# Autodesk Inventor assembly: Prototype-Chassis-1
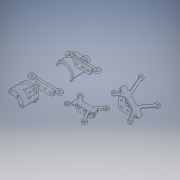
[picture p0: Inventor's stored thumbnail of the model, 180x180]
Saved by Autodesk Inventor 2017 (Build 210142000, 142)
## iProperties
Created: 2018-04-11
Part Number: Prototype-Chassis-1
Document SubType Name: Assembly
Designer: MtgSaber
Author: MtgSaber
## Documents named in this file (12)
- D:\Programming\Projects\Pirover\autodesk\Prototype-Chassis-1.iam
- D:\Programming\Projects\Pirover\autodesk\2.5in-wheel\2.5in-Wheel-2.ipt
- D:\Programming\Projects\Pirover\autodesk\Nextrox-Mini-12VDC-60rpmGearbox-Motor\Nextrox-Mini-12VDC-60rpmGearbox-Motor.ipt
- D:\Programming\Projects\Pirover\autodesk\Keystone-26650-Dual-Battery-Holder\Keystone-26650-Dual-Battery-Holder[DWG-1109].ipt
- D:\Programming\Projects\Pirover\autodesk\Drok-DC-9v+-to-5v-Converter\Drok-DC-9v+-to-5v-Converter.ipt
- D:\Programming\Projects\Pirover\autodesk\Raspberry-Pi-3BPlus[with_Screen]\Raspberry-Pi-3B[with_Screen].ipt
- D:\Programming\Projects\Pirover\autodesk\Arduino-Uno-r3\Arduino-Uno-r3.ipt
- D:\Programming\Projects\Pirover\autodesk\ChasssiPrototypeA2.ipt
- D:\Programming\Projects\Pirover\autodesk\ChasssiPrototypeA2_MIR.ipt
- D:\Programming\Projects\Pirover\autodesk\ChassisPrototypeA3.ipt
- D:\Programming\Projects\Pirover\autodesk\ChassisPrototypeA4.ipt
- D:\Programming\Projects\Pirover\autodesk\ChassisPrototypeA5.ipt
## Components (15 placed, 11 different names)
1. Nextrox-Mini-12VDC-60rpmGearbox-Motor:1 — Mate:2, Mate:3, Mate:9, Flush:11, Flush:15, Mate:17, Mate:18, Mate:20, Mate:21, Mate:22
2. Nextrox-Mini-12VDC-60rpmGearbox-Motor:2 — Mate:2, Mate:3, Flush:10, Flush:14, Mate:15, Mate:16, Mate:19, Flush:16
3. Keystone-26650-Dual-Battery-Holder[DWG-1109]:1 — Mate:5, Flush:2, Flush:3, Mate:6, Flush:7, Flush:8, Mate:7, Flush:11, Flush:12, Mate:23, Mate:24
4. Keystone-26650-Dual-Battery-Holder[DWG-1109]:2 — Mate:5, Flush:2, Flush:3, Flush:6, Flush:10, Mate:19, Flush:17, Flush:18
5. Drok-DC-9v+-to-5v-Converter:1 — Flush:1, Flush:5, Mate:6, Flush:7, Mate:12
6. Raspberry-Pi-3B[with_Screen]:1 — Flush:13, Mate:11, Angle:1, Mate:13, Angle:2, Flush:26, Flush:27
7. Arduino-Uno-r3:1 — Flush:1, Flush:5, Flush:6, Mate:8, Flush:21, Flush:22, Flush:23, Flush:24, Flush:25
8. 2.5in-Wheel-2:1 — Flush:15, Mate:17, Mate:18
9. 2.5in-Wheel-2:2 — Flush:14, Mate:15, Mate:16
10. ChasssiPrototypeA2:1 — Flush:16
11. ChasssiPrototypeA2_MIR:1 — Mate:20, Mate:21, Mate:22
12. ChassisPrototypeA3:1 — Flush:17, Flush:19, Flush:20
13. ChassisPrototypeA3:2 — Mate:23, Flush:20, Mate:24
14. ChassisPrototypeA4:1 — Flush:21, Flush:23, Flush:24, Flush:25
15. ChassisPrototypeA5:1 — Flush:26, Flush:28
## Relationships (49: Flush 26, Mate 21, Angle 2)
- Mate:2: Nextrox-Mini-12VDC-60rpmGearbox-Motor:1 ↔ Nextrox-Mini-12VDC-60rpmGearbox-Motor:2
- Mate:3: Nextrox-Mini-12VDC-60rpmGearbox-Motor:1 ↔ Nextrox-Mini-12VDC-60rpmGearbox-Motor:2
- Flush:1: Drok-DC-9v+-to-5v-Converter:1 ↔ Arduino-Uno-r3:1
- Mate:5 (25.4 mm): Keystone-26650-Dual-Battery-Holder[DWG-1109]:1 ↔ Keystone-26650-Dual-Battery-Holder[DWG-1109]:2
- Flush:2: Keystone-26650-Dual-Battery-Holder[DWG-1109]:1 ↔ Keystone-26650-Dual-Battery-Holder[DWG-1109]:2
- Flush:3: Keystone-26650-Dual-Battery-Holder[DWG-1109]:1 ↔ Keystone-26650-Dual-Battery-Holder[DWG-1109]:2
- Flush:5: Drok-DC-9v+-to-5v-Converter:1 ↔ Arduino-Uno-r3:1
- Mate:6 (25.4 mm): Keystone-26650-Dual-Battery-Holder[DWG-1109]:1 ↔ Drok-DC-9v+-to-5v-Converter:1
- Flush:6: Keystone-26650-Dual-Battery-Holder[DWG-1109]:2 ↔ Arduino-Uno-r3:1
- Flush:7: Keystone-26650-Dual-Battery-Holder[DWG-1109]:1 ↔ Drok-DC-9v+-to-5v-Converter:1
- Flush:8: Keystone-26650-Dual-Battery-Holder[DWG-1109]:1
- Mate:7: Keystone-26650-Dual-Battery-Holder[DWG-1109]:1
- Mate:8: Arduino-Uno-r3:1
- Mate:9 (-38.1 mm): Nextrox-Mini-12VDC-60rpmGearbox-Motor:1
- Flush:10: Nextrox-Mini-12VDC-60rpmGearbox-Motor:2 ↔ Keystone-26650-Dual-Battery-Holder[DWG-1109]:2
- Flush:11: Nextrox-Mini-12VDC-60rpmGearbox-Motor:1 ↔ Keystone-26650-Dual-Battery-Holder[DWG-1109]:1
- Flush:12 (12.7 mm): Keystone-26650-Dual-Battery-Holder[DWG-1109]:1
- Flush:13: Raspberry-Pi-3B[with_Screen]:1
- Mate:11: Raspberry-Pi-3B[with_Screen]:1
- Angle:1 (-45 deg): Raspberry-Pi-3B[with_Screen]:1
- Mate:12 (25.4 mm): Drok-DC-9v+-to-5v-Converter:1
- Mate:13: Raspberry-Pi-3B[with_Screen]:1
- Angle:2 (45 deg): Raspberry-Pi-3B[with_Screen]:1
- Mate:14
- Flush:14: Nextrox-Mini-12VDC-60rpmGearbox-Motor:2 ↔ 2.5in-Wheel-2:2
- Mate:15: Nextrox-Mini-12VDC-60rpmGearbox-Motor:2 ↔ 2.5in-Wheel-2:2
- Mate:16: Nextrox-Mini-12VDC-60rpmGearbox-Motor:2 ↔ 2.5in-Wheel-2:2
- Flush:15: Nextrox-Mini-12VDC-60rpmGearbox-Motor:1 ↔ 2.5in-Wheel-2:1
- Mate:17: Nextrox-Mini-12VDC-60rpmGearbox-Motor:1 ↔ 2.5in-Wheel-2:1
- Mate:18: Nextrox-Mini-12VDC-60rpmGearbox-Motor:1 ↔ 2.5in-Wheel-2:1
- Mate:19: Nextrox-Mini-12VDC-60rpmGearbox-Motor:2 ↔ Keystone-26650-Dual-Battery-Holder[DWG-1109]:2
- Flush:16: Nextrox-Mini-12VDC-60rpmGearbox-Motor:2 ↔ ChasssiPrototypeA2:1
- Mate:20: Nextrox-Mini-12VDC-60rpmGearbox-Motor:1 ↔ ChasssiPrototypeA2_MIR:1
- Mate:21: Nextrox-Mini-12VDC-60rpmGearbox-Motor:1 ↔ ChasssiPrototypeA2_MIR:1
- Mate:22: Nextrox-Mini-12VDC-60rpmGearbox-Motor:1 ↔ ChasssiPrototypeA2_MIR:1
- Flush:17: Keystone-26650-Dual-Battery-Holder[DWG-1109]:2 ↔ ChassisPrototypeA3:1
- Flush:18 (-27.94 mm): Keystone-26650-Dual-Battery-Holder[DWG-1109]:2
- Flush:19: ChassisPrototypeA3:1
- Mate:23: Keystone-26650-Dual-Battery-Holder[DWG-1109]:1 ↔ ChassisPrototypeA3:2
- Flush:20: ChassisPrototypeA3:1 ↔ ChassisPrototypeA3:2
- Mate:24: Keystone-26650-Dual-Battery-Holder[DWG-1109]:1 ↔ ChassisPrototypeA3:2
- Flush:21: Arduino-Uno-r3:1 ↔ ChassisPrototypeA4:1
- Flush:22 (3.175 mm): Arduino-Uno-r3:1
- Flush:23 (3.175 mm): Arduino-Uno-r3:1 ↔ ChassisPrototypeA4:1
- Flush:24: Arduino-Uno-r3:1 ↔ ChassisPrototypeA4:1
- Flush:25: Arduino-Uno-r3:1 ↔ ChassisPrototypeA4:1
- Flush:26: Raspberry-Pi-3B[with_Screen]:1 ↔ ChassisPrototypeA5:1
- Flush:27 (-42.4942 mm): Raspberry-Pi-3B[with_Screen]:1
- Flush:28: ChassisPrototypeA5:1
